# Autodesk Inventor assembly: DoorLockAssembly
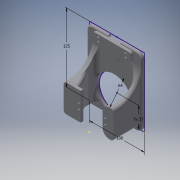
[picture p0: Inventor's stored thumbnail of the model, 180x180]
Saved by Autodesk Inventor 2019 (Build 230136000, 136)
## iProperties
Created: 2019-05-08
Part Number: DoorLockAssembly
Document SubType Name: Assembly
Designer: Iván
Author: Iván
## Documents named in this file (3)
- C:\Users\Iván\Documents\Github\DoorLock\LockSupport\DoorLockAssembly.iam
- C:\Users\Iván\Documents\Github\DoorLock\LockSupport\RotationLock.ipt
- C:\Users\Iván\Documents\Github\DoorLock\LockSupport\DoorLockSupport.ipt
## Components (2 placed, 2 different names)
1. DoorLockSupport:1 — Mate:1, Mate:2, Mate:3
2. RotationLock:1 — Mate:1, Mate:2, Mate:3
## Relationships (3: Mate 3)
- Mate:1: DoorLockSupport:1 ↔ RotationLock:1
- Mate:2: DoorLockSupport:1 ↔ RotationLock:1
- Mate:3: DoorLockSupport:1 ↔ RotationLock:1
